# Autodesk Inventor assembly: Flywheel
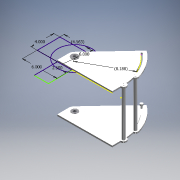
[picture p0: Inventor's stored thumbnail of the model, 180x180]
Saved by Autodesk Inventor 2018.3 (Build 223284000, 284)
## iProperties
Created: 2020-01-19
Part Number: Flywheel
Document SubType Name: Assembly
Designer: Victor
Author: Victor
## Documents named in this file (6)
- C:\Users\22barlalex\Documents\GrabCAD\Infinite Recharge 2020\Build season\Flywheel\FLY_000_Flywheel.iam
- C:\Users\22barlalex\Documents\GrabCAD\Infinite Recharge 2020\Build season\Flywheel\FLY_003_HoodRod.ipt
- C:\Users\22barlalex\Documents\GrabCAD\Infinite Recharge 2020\Build season\Flywheel\0_500_ID_x_1_125_OD_x_0_313_WD_Flanged_Bearing_217-2731.ipt
- C:\Users\22barlalex\Documents\GrabCAD\Infinite Recharge 2020\Build season\Flywheel\FLY_002_HoodPanelRight.ipt
- C:\Users\22barlalex\Documents\GrabCAD\Infinite Recharge 2020\Build season\Flywheel\FLY_001_HoodPanelLeft.ipt
- E:\Downloads\GrabCAD\Deep Space 2019\Build Season\CLB_Rear_Motor.iam
## Components (8 placed, 5 different names)
1. FLY_003_HoodRod:1 — Insert:4, Insert:7
2. FLY_003_HoodRod:4 — Insert:2, Insert:8
3. 0_500_ID_x_1_125_OD_x_0_313_WD_Flanged_Bearing_217-2731:1 — Insert:9
4. 0_500_ID_x_1_125_OD_x_0_313_WD_Flanged_Bearing_217-2731:2 — Insert:10
5. FLY_002_HoodPanelRight:1 — Insert:2, Insert:4, Insert:10
6. FLY_001_HoodPanelLeft:1 — Insert:7, Insert:8, Insert:9
7. CLB_Rear_Motor:1 [sub-assembly]
8. CLB_Rear_Motor:2 [sub-assembly]
## Relationships (6: Insert 6)
- Insert:2: FLY_003_HoodRod:4 ↔ FLY_002_HoodPanelRight:1
- Insert:4: FLY_003_HoodRod:1 ↔ FLY_002_HoodPanelRight:1
- Insert:7: FLY_003_HoodRod:1 ↔ FLY_001_HoodPanelLeft:1
- Insert:8: FLY_003_HoodRod:4 ↔ FLY_001_HoodPanelLeft:1
- Insert:9: 0_500_ID_x_1_125_OD_x_0_313_WD_Flanged_Bearing_217-2731:1 ↔ FLY_001_HoodPanelLeft:1
- Insert:10: 0_500_ID_x_1_125_OD_x_0_313_WD_Flanged_Bearing_217-2731:2 ↔ FLY_002_HoodPanelRight:1
